# Autodesk Inventor assembly: X_CarriageL_V2_1_Short
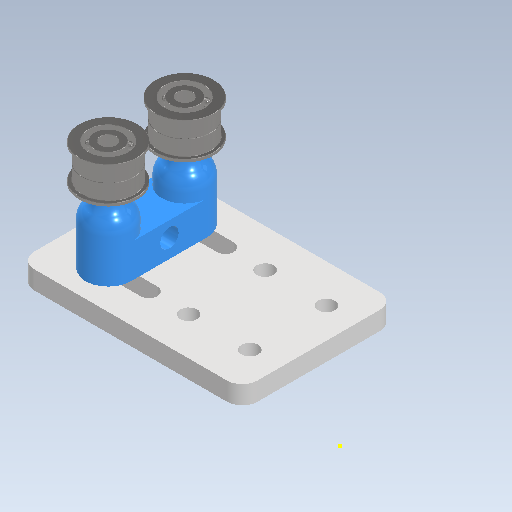
[picture p0: Inventor's stored thumbnail of the model, 512x512]
Saved by Autodesk Inventor 2021 (Build 250183000, 183)
## iProperties
Created: 2021-06-13
Part Number: X_CarriageL_V2_1_Short
Document SubType Name: Assembly
Designer: Jorian Brusind
Author: Jorian Brusind
## Documents named in this file (5)
- C:\Users\Jorian Brusind\Documents\GitHub\HyperRail\Inventor Files\X_CarriageL_V2_1_Short.iam
- C:\Users\Jorian Brusind\Documents\GitHub\HyperRail\Inventor Files\4mm_Roller_Spacer_simple.ipt
- C:\Users\Jorian Brusind\Documents\GitHub\HyperRail\Inventor Files\X_Carriage_Plate_Short.ipt
- C:\Users\Jorian Brusind\Documents\GitHub\HyperRail\Inventor Files\miniature-ball-bearings-metric-series-flanged-1.snapshot.1\F606ZZFlanged\F608 - 8 x 22 x 7.ipt
- C:\Users\Jorian Brusind\Documents\GitHub\PersonalProjects\HyperRail\Inventor Files\miniature-ball-bearings-metric-series-flanged-1.snapshot.1\F606ZZFlanged.ipt
## Components (6 placed, 3 different names)
1. X_Carriage_Plate_Short:1 — Mate:6, Mate:7, Angle:1
2. 4mm_Roller_Spacer_simple:1 — Mate:6, Mate:7, Angle:1, Mate:8, Mate:9, Mate:13
3. F608 - 8 x 22 x 7:1 — Mate:8, Mate:10, Flush:2, Mate:12, Mate:13
4. F608 - 8 x 22 x 7:2 — Mate:11, Flush:1
5. F608 - 8 x 22 x 7:3 — Mate:9, Mate:11, Flush:2
6. F608 - 8 x 22 x 7:4 — Mate:10, Flush:1, Mate:12
## Relationships (11: Mate 8, Flush 2, Angle 1)
- Mate:6: X_Carriage_Plate_Short:1 ↔ 4mm_Roller_Spacer_simple:1
- Mate:7 (-12.5 mm): X_Carriage_Plate_Short:1 ↔ 4mm_Roller_Spacer_simple:1
- Angle:1 (0 deg): X_Carriage_Plate_Short:1 ↔ 4mm_Roller_Spacer_simple:1
- Mate:8: 4mm_Roller_Spacer_simple:1 ↔ F608 - 8 x 22 x 7:1
- Mate:9: 4mm_Roller_Spacer_simple:1 ↔ F608 - 8 x 22 x 7:3
- Mate:10: F608 - 8 x 22 x 7:1 ↔ F608 - 8 x 22 x 7:4
- Mate:11: F608 - 8 x 22 x 7:2 ↔ F608 - 8 x 22 x 7:3
- Flush:1: F608 - 8 x 22 x 7:2 ↔ F608 - 8 x 22 x 7:4
- Flush:2: F608 - 8 x 22 x 7:1 ↔ F608 - 8 x 22 x 7:3
- Mate:12: F608 - 8 x 22 x 7:1 ↔ F608 - 8 x 22 x 7:4
- Mate:13: 4mm_Roller_Spacer_simple:1 ↔ F608 - 8 x 22 x 7:1
